# Autodesk Inventor assembly: eye-to-body
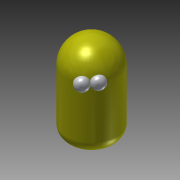
[picture p0: Inventor's stored thumbnail of the model, 180x180]
Saved by Autodesk Inventor 2015 (Build 190159000, 159)
## iProperties
Created: 2014-12-10
Part Number: eye-to-body
Document SubType Name: Assembly
Designer: joe
Author: joe
## Documents named in this file (3)
- C:\Users\joe\Desktop\minion-design\eye-to-body.iam
- C:\Users\joe\Desktop\minion-design\minion-body.ipt
- C:\Users\joe\Desktop\minion-design\minion-eye.ipt
## Components (3 placed, 2 different names)
1. minion-body:1 — Tangent:1
2. minion-eye:1 — Tangent:1
3. minion-eye:2
## Relationships (1: Tangent 1)
- Tangent:1: minion-body:1 ↔ minion-eye:1
